# Autodesk Inventor assembly: MaxonEC45-50W-MILE-Machined-with-gear
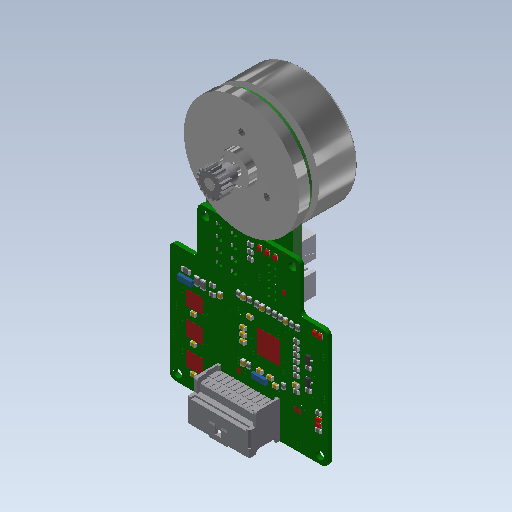
[picture p0: Inventor's stored thumbnail of the model, 512x512]
Saved by Autodesk Inventor 2020.2 (Build 242310000, 310)
## iProperties
Created: 2015-08-10
Part Number: MaxonEC45-50W-MILE-Machined-with-gear
Document SubType Name: Assembly
Designer: ryll
Author: ryll
## Documents named in this file (6)
- C:\Users\Acer\Fusion\RobôCIn\SSL\2020_LARC\FIRST_FLOOR\Motor\MaxonEC45-50W-MILE-Machined-with-gear.iam
- C:\Users\Acer\Fusion\RobôCIn\SSL\2020_LARC\first_floor\Motor\MaxonEC45-50W-MILE.ipt
- C:\Users\Acer\Fusion\RobôCIn\SSL\2020_LARC\first_floor\Motor\IDC Stecker 10pol.ipt
- C:\Users\Acer\Fusion\RobôCIn\SSL\2020_LARC\first_floor\Motor\Molex MiniFit 8pol.ipt
- C:\Users\Acer\Fusion\RobôCIn\SSL\2020_LARC\first_floor\Motor\gear_z18_21101800(modified).ipt
- C:\Users\Acer\Fusion\RobôCIn\SSL\2020_LARC\first_floor\Components\MotorBoard\MOTORBOARD_V1.0.IAM
## Components (5 placed, 5 different names)
1. MaxonEC45-50W-MILE:1 — Passend:1, Passend:2, Fluchtend:1, Fluchtend:2, Fluchtend:3, Fluchtend:4, Mate:3, Mate:4, Mate:5, Mate:6, Mate:7
2. IDC Stecker 10pol:1 — Passend:2, Fluchtend:1, Fluchtend:2
3. Molex MiniFit 8pol:1 — Passend:1, Fluchtend:3, Fluchtend:4
4. Ritzel z=18:1 — Mate:3, Mate:4
5. MOTORBOARD_V1.0:1 [sub-assembly] — Mate:5, Mate:6, Mate:7
## Relationships (11: Mate 7, Flush 4)
- Passend:1 [Mate]: MaxonEC45-50W-MILE:1 ↔ Molex MiniFit 8pol:1
- Passend:2 [Mate]: MaxonEC45-50W-MILE:1 ↔ IDC Stecker 10pol:1
- Fluchtend:1 [Flush] (2 mm): MaxonEC45-50W-MILE:1 ↔ IDC Stecker 10pol:1
- Fluchtend:2 [Flush] (4 mm): MaxonEC45-50W-MILE:1 ↔ IDC Stecker 10pol:1
- Fluchtend:3 [Flush] (4 mm): MaxonEC45-50W-MILE:1 ↔ Molex MiniFit 8pol:1
- Fluchtend:4 [Flush] (4 mm): MaxonEC45-50W-MILE:1 ↔ Molex MiniFit 8pol:1
- Mate:3: MaxonEC45-50W-MILE:1 ↔ Ritzel z=18:1
- Mate:4 (1 mm): MaxonEC45-50W-MILE:1 ↔ Ritzel z=18:1
- Mate:5: MaxonEC45-50W-MILE:1 ↔ MOTORBOARD_V1.0:1
- Mate:6 (-22.5 mm): MaxonEC45-50W-MILE:1 ↔ MOTORBOARD_V1.0:1
- Mate:7 (-37.25 mm): MaxonEC45-50W-MILE:1 ↔ MOTORBOARD_V1.0:1
